# Autodesk Inventor assembly: SingleCrossover_Curve
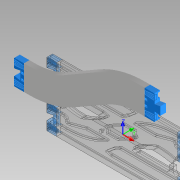
[picture p0: Inventor's stored thumbnail of the model, 180x180]
Saved by Autodesk Inventor 2021 (Build 250183000, 183)
## iProperties
Created: 2021-03-17
Part Number: SingleCrossover_Curve
Document SubType Name: Assembly
Designer: kumagai
Author: kumagai
## Documents named in this file (6)
- X:\Develop\CAD\PlaRails\Crossover\SingleCrossoverIA_MIR\SingleCrossover_Curve.iam
- X:\Develop\CAD\PlaRails\RailJointFemale.ipt
- X:\Develop\CAD\PlaRails\RailJointMale.ipt
- X:\Develop\CAD\PlaRails\GlobalParameter.ipt
- X:\Develop\CAD\PlaRails\Crossover\SingleCross_CurveHalf_MIR.ipt
- X:\Develop\CAD\PlaRails\Crossover\SingleCrossoverIA_MIR.iam
## Components (4 placed, 3 different names)
1. SingleCross_CurveHalf_MIR:1
2. SingleCross_CurveHalf_MIR:2
3. RailJointFemale:2 — フラッシュ:6, フラッシュ:8, フラッシュ:10
4. RailJointMale:1 — フラッシュ:11, フラッシュ:13, フラッシュ:15
## Relationships (12: Flush 10, Mate 2)
- フラッシュ:6 [Flush] (-5.2 mm): RailJointFemale:2
- フラッシュ:8 [Flush] (-30 mm): RailJointFemale:2
- フラッシュ:10 [Flush] (-92.5 mm): RailJointFemale:2
- フラッシュ:11 [Flush] (-5.2 mm): RailJointMale:1
- フラッシュ:13 [Flush] (30 mm): RailJointMale:1
- フラッシュ:15 [Flush] (92.5 mm): RailJointMale:1
- [Flush]: SingleCross_CurveHalf_MIR:1
- [Flush]: SingleCross_CurveHalf_MIR:1
- [Flush]: SingleCross_CurveHalf_MIR:1
- [Flush]: SingleCross_CurveHalf_MIR:2
- [Mate]: SingleCross_CurveHalf_MIR:2
- [Mate]: SingleCross_CurveHalf_MIR:2
## Named parameters: PrinterOffset = 0 mm, StraightLength = 215 mm, RailWidth = 38 mm, OuterWall = 2 mm, InnerWall = 2.4 mm, InsideWidth = 18.6 mm, RailHeight = 8.4 mm, RailDepth = 3.2 mm, ConnectorLength = 15 mm, JointMW1 = 13 mm, JointMW2 = 9.4 mm, JointMH = 9 mm, JointFW1 = 13.3 mm, JointFW2 = 9.6 mm, JointFH = 9.5 mm, DoubleWidth = 60 mm, ViaductHeight = 66 mm, SupportGap = 0.2 mm, SupportRib = 0.5 mm
